# Autodesk Inventor assembly: 0226_OmniB
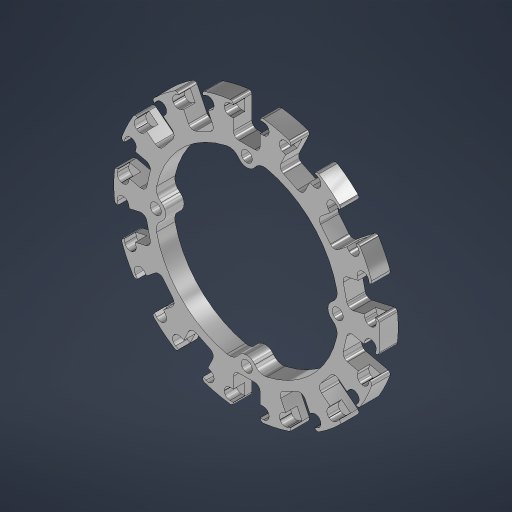
[picture p0: Inventor's stored thumbnail of the model, 512x512]
Saved by Autodesk Inventor 2024.2 (Build 282272000, 272)
## iProperties
Created: 2024-02-26
Part Number: 0226_OmniB
Document SubType Name: Assembly
Designer: Hanaoka
Author: Hanaoka
## Documents named in this file (2)
- G:\共有ドライブ\reRo\05_個人\hanaoka\inventor\DribblerUnit\0226_OmniB.iam
- G:\共有ドライブ\reRo\05_個人\hanaoka\inventor\DriveUnit\OmniFrame_B.ipt
## Components (1 placed, 1 different names)
1. OmniFrame_B:1 — メイト:1, メイト:2, 正接:1
## Relationships (3: Mate 2, Tangent 1)
- メイト:1 [Mate]: OmniFrame_B:1
- メイト:2 [Mate] (6 mm): OmniFrame_B:1
- 正接:1 [Tangent]: OmniFrame_B:1
